# Autodesk Inventor assembly: 6_right_arm_no error
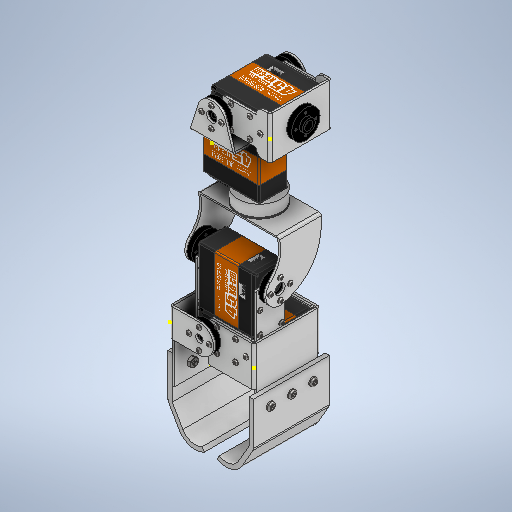
[picture p0: Inventor's stored thumbnail of the model, 512x512]
Saved by Autodesk Inventor 2026.1 (Build 301233000, 233)
## iProperties
Created: 2025-07-28
Part Number: 6_right_arm_no error
Document SubType Name: Assembly
Designer: LG
Author: LG
## Documents named in this file (20)
- C:\Users\LG\Desktop\RHp_Humanoid_ver1\Assembly\6_right_Arm.iam
- C:\Users\LG\Desktop\RHp_Humanoid_ver1\Part\HTD-45H, Horn\HTD-45H\HTD-45H.iam
- C:\Users\LG\Desktop\RHp_Humanoid_ver1\Part\HTD-45H, Horn\Horn\Top Horn.ipt
- C:\Users\LG\Desktop\RHp_Humanoid_ver1\Part\Frame\Arm\axis_18_top_frame.ipt
- C:\Users\LG\Desktop\RHp_Humanoid_ver1\Part\HTD-45H, Horn\Horn\Bottom Horn.ipt
- C:\Users\LG\Desktop\RHp_Humanoid_ver1\Part\Frame\Arm\axis_19_bottom_frame.ipt
- C:\Users\LG\Desktop\RHp_Humanoid_ver1\Part\Frame\Arm\axis_20_top_frame.ipt
- C:\Users\LG\Desktop\RHp_Humanoid_ver1\Part\Bolt, Bearing, Nut, Washer\2030 Teflon Sheet.ipt
- C:\Users\LG\Desktop\RHp_Humanoid_ver1\Part\Frame\Arm\axis_20_bottom_frame.ipt
- C:\Users\LG\Desktop\RHp_Humanoid_ver1\Part\Frame\Arm\axis_21_top_frame.ipt
- C:\Users\LG\Desktop\RHp_Humanoid_ver1\Part\Frame\Arm\axis_21_bottom_frame.ipt
- C:\Users\LG\Desktop\RHp_Humanoid_ver1\Part\Frame\Arm\axis_22_bottom_frame.ipt
- C:\Users\LG\Desktop\RHp_Humanoid_ver1\Part\Frame\Arm\axis_22_top_frame.ipt
- C:\Users\LG\Desktop\RHp_Humanoid_ver1\Part\Frame\Arm\HTD-45H_no bottom horn.ipt
- C:\Users\LG\Desktop\RHp_Humanoid_ver1\Part\Frame\Arm\gripper_frame.ipt
- C:\Users\LG\Desktop\RHp_Humanoid_ver1\Part\Bolt, Bearing, Nut, Washer\볼트, 너트\M2x4 Bolt.ipt
- C:\Users\LG\Desktop\RHp_Humanoid_ver1\Part\Bolt, Bearing, Nut, Washer\볼트, 너트\M3x6 Bolt.ipt
- C:\Users\LG\Desktop\RHp_Humanoid_ver1\Part\Bolt, Bearing, Nut, Washer\볼트, 너트\M3 Nut.ipt
- C:\Users\LG\Desktop\RHp_Humanoid_ver1\Part\Bolt, Bearing, Nut, Washer\볼트, 너트\M2x6 Bolt.ipt
- C:\Users\LG\Desktop\RHp_Humanoid_ver1\Part\Bolt, Bearing, Nut, Washer\볼트, 너트\M3x8 Bolt.ipt
## Components (107 placed, 18 different names)
1. M2x4 Bolt:21 — Rigid:22
2. M2x4 Bolt:20 — Rigid:21
3. M2x4 Bolt:19 — Rigid:20
4. M2x4 Bolt:18 — Rigid:19
5. M2x4 Bolt:6 — Rigid:6
6. M2x4 Bolt:8 — Rigid:2
7. M2x4 Bolt:7 — Rigid:3
8. M2x4 Bolt:9 — Rigid:4
9. M2x4 Bolt:1 — Rigid:5
10. M2x4 Bolt:10 — Rigid:12
11. M2x4 Bolt:11 — Rigid:13
12. M2x4 Bolt:17 — Rigid:11
13. M2x4 Bolt:16 — Rigid:14
14. axis_18_top_frame:1 — Mate:6, Mate:7, Mate:8, Mate:9, Mate:14, Mate:15, Rigid:2, Rigid:3, Rigid:4, Rigid:5, Rigid:6, Rigid:11, Rigid:12, Rigid:13, Rigid:14, Rigid:19, Rigid:20, Rigid:21, Rigid:22
15. Top Horn:1 — Mate:6, Mate:14, Mate:15
16. M2x4 Bolt:2 — Rigid:7
17. M2x4 Bolt:4 — Rigid:9
18. M2x4 Bolt:5 — Rigid:8
19. M2x4 Bolt:3 — Rigid:10
20. M2x4 Bolt:13 — Rigid:15
21. M2x4 Bolt:12 — Rigid:17
22. M2x4 Bolt:15 — Rigid:18
23. M2x4 Bolt:14 — Rigid:16
24. M2x4 Bolt:55 — Rigid:96
25. M2x4 Bolt:56 — Rigid:98
26. M2x4 Bolt:57 — Rigid:95
27. M2x4 Bolt:58 — Rigid:97
28. axis_19_bottom_frame:1 — Flush:2, Mate:12, Mate:13, Rigid:7, Rigid:8, Rigid:9, Rigid:10, Rigid:15, Rigid:16, Rigid:17, Rigid:18, Mate:49, Mate:50, Flush:15, Rigid:95, Rigid:96, Rigid:97, Rigid:98
29. Bottom Horn:1 — Mate:10, Mate:11, Flush:1
30. Top Horn:2 — Rotational:2, Flush:2, Mate:12, Mate:13
31. HTD-45H:2 [sub-assembly] — Mate:7, Mate:8, Mate:9, Rotational:2, Mate:10, Mate:11, Flush:1
32. 2030 Teflon Sheet:1 — Mate:19, Mate:20, Mate:21, Mate:24, Mate:25
33. 2030 Teflon Sheet:2 — Mate:24, Mate:25, Mate:26
34. M2x4 Bolt:27 — Rigid:27
35. M2x4 Bolt:28 — Rigid:29
36. M2x4 Bolt:29 — Rigid:30
37. M2x4 Bolt:26 — Rigid:28
38. axis_20_top_frame:1 — Mate:19, Mate:20, Mate:21, Mate:47, Flush:14, Mate:48
39. axis_20_bottom_frame:1 — Mate:22, Flush:6, Mate:23, Mate:26, Mate:29, Mate:30, Mate:31, Rigid:27, Rigid:28, Rigid:29, Rigid:30, Rigid:31, Rigid:32, Rigid:33, Rigid:34, Rigid:35, Rigid:36, Rigid:37, Rigid:38
40. Top Horn:3 — Mate:22, Flush:6, Mate:23, Rotational:6
41. HTD-45H:6 — Rotational:6, Mate:47, Flush:14, Mate:48, Mate:49, Mate:50, Flush:15
42. M2x4 Bolt:30 — Rigid:31
43. M2x4 Bolt:31 — Rigid:32
44. M2x4 Bolt:33 — Rigid:33
45. M2x4 Bolt:32 — Rigid:34
46. M2x4 Bolt:34 — Rigid:35
47. M2x4 Bolt:35 — Rigid:37
48. M2x4 Bolt:36 — Rigid:36
49. M2x4 Bolt:37 — Rigid:38
50. M2x4 Bolt:43 — Rigid:44
51. M2x4 Bolt:44 — Rigid:45
52. M2x4 Bolt:45 — Rigid:46
53. M2x4 Bolt:46 — Rigid:47
54. M2x4 Bolt:39 — Rigid:40
55. M2x4 Bolt:38 — Rigid:39
56. M2x4 Bolt:41 — Rigid:42
57. M2x4 Bolt:40 — Rigid:41
58. M2x4 Bolt:42 — Rigid:43
59. M3 Nut:3 — Rigid:64
60. M3 Nut:4 — Rigid:62
61. M3 Nut:2 — Rigid:63
62. M3 Nut:1 — Rigid:61
63. M3x6 Bolt:1 — Rigid:58
64. M3x6 Bolt:2 — Rigid:59
65. M3x6 Bolt:3 — Rigid:60
66. M3x6 Bolt:4 — Rigid:57
67. axis_21_top_frame:1 — Mate:36, Mate:37, Mate:38, Mate:39, Mate:45, Rigid:39, Rigid:40, Rigid:41, Rigid:42, Rigid:43, Rigid:44, Rigid:45, Rigid:46, Rigid:47, Rigid:57, Rigid:58, Rigid:59, Rigid:60
68. axis_21_bottom_frame:1 — Mate:39, Mate:40, Flush:10, Mate:44, Flush:11, Rigid:61, Rigid:62, Rigid:63, Rigid:64
69. Bottom Horn:2 — Mate:27, Flush:7, Mate:28
70. Top Horn:4 — Rotational:4, Mate:29, Mate:30, Mate:31
71. HTD-45H:4 [sub-assembly] — Mate:27, Flush:7, Mate:28, Rotational:4, Mate:35, Flush:8, Flush:9, Mate:37, Mate:38
72. M2x4 Bolt:47 — Rigid:65
73. M2x4 Bolt:49 — Rigid:66
74. M2x4 Bolt:50 — Rigid:68
75. M2x4 Bolt:48 — Rigid:67
76. M2x4 Bolt:54 — Rigid:69
77. M2x4 Bolt:51 — Rigid:70
78. M2x4 Bolt:53 — Rigid:72
79. M2x4 Bolt:52 — Rigid:71
80. M2x6 Bolt:5 — Rigid:77
81. M2x6 Bolt:7 — Rigid:78
82. M2x6 Bolt:6 — Rigid:79
83. M2x6 Bolt:8 — Rigid:80
84. M2x6 Bolt:9 — Rigid:81
85. M2x6 Bolt:2 — Rigid:74
86. M2x6 Bolt:1 — Rigid:73
87. M2x6 Bolt:3 — Rigid:76
88. M2x6 Bolt:4 — Rigid:75
89. M3x8 Bolt:4 — Rigid:88
90. M3x8 Bolt:5 — Rigid:89
91. M3x8 Bolt:6 — Rigid:90
92. M3 Nut:10 — Rigid:93
93. M3 Nut:9 — Rigid:92
94. M3 Nut:8 — Rigid:91
95. M3x8 Bolt:3 — Rigid:84
96. M3x8 Bolt:2 — Rigid:83
97. M3x8 Bolt:1 — Rigid:82
98. M3 Nut:6 — Rigid:87
99. M3 Nut:7 — Rigid:86
100. M3 Nut:5 — Rigid:85
101. axis_22_bottom_frame:1 — Mate:41, Mate:42, Mate:43, Rigid:1, Rigid:65, Rigid:66, Rigid:67, Rigid:68, Rigid:69, Rigid:70, Rigid:71, Rigid:72, Rigid:85, Rigid:86, Rigid:87
102. axis_22_top_frame:1 — Mate:44, Flush:11, Mate:45, Rigid:73, Rigid:74, Rigid:75, Rigid:76, Rigid:77, Rigid:78, Rigid:79, Rigid:80, Rigid:81, Rigid:91, Rigid:92, Rigid:93, Rigid:94
103. gripper_frame:1 — Rigid:1, Rigid:82, Rigid:83, Rigid:84
104. gripper_frame:2 — Rigid:88, Rigid:89, Rigid:90, Rigid:94
105. Top Horn:5 — Rotational:5, Mate:41, Mate:42, Mate:43
106. Bottom Horn:3 — Mate:32, Mate:33, Mate:34
107. HTD-45H:5 [sub-assembly] — Rotational:5, Mate:32, Mate:33, Mate:34, Mate:35, Flush:8, Flush:9, Mate:36, Mate:40, Flush:10
## Relationships (140: WeldJoint 85, Mate 41, Flush 10, RevoluteJoint 4)
- Rotational:2 [RevoluteJoint]: Top Horn:2 ↔ HTD-45H:2
- Rotational:4 [RevoluteJoint]: Top Horn:4 ↔ HTD-45H:4
- Rotational:5 [RevoluteJoint]: Top Horn:5 ↔ HTD-45H:5
- Rotational:6 [RevoluteJoint]: Top Horn:3 ↔ HTD-45H:6
- Mate:6: axis_18_top_frame:1 ↔ Top Horn:1
- Mate:7: axis_18_top_frame:1 ↔ HTD-45H:2
- Mate:8 (2.5 mm): axis_18_top_frame:1 ↔ HTD-45H:2
- Mate:9: axis_18_top_frame:1 ↔ HTD-45H:2
- Mate:10: Bottom Horn:1 ↔ HTD-45H:2
- Mate:11: Bottom Horn:1 ↔ HTD-45H:2
- Flush:1: Bottom Horn:1 ↔ HTD-45H:2
- Flush:2 (14.5 mm): axis_19_bottom_frame:1 ↔ Top Horn:2
- Mate:12: axis_19_bottom_frame:1 ↔ Top Horn:2
- Mate:13: axis_19_bottom_frame:1 ↔ Top Horn:2
- Mate:14: axis_18_top_frame:1 ↔ Top Horn:1
- Mate:15: axis_18_top_frame:1 ↔ Top Horn:1
- Mate:19: 2030 Teflon Sheet:1 ↔ axis_20_top_frame:1
- Mate:20: 2030 Teflon Sheet:1 ↔ axis_20_top_frame:1
- Mate:21: 2030 Teflon Sheet:1 ↔ axis_20_top_frame:1
- Mate:22: axis_20_bottom_frame:1 ↔ Top Horn:3
- Flush:6: axis_20_bottom_frame:1 ↔ Top Horn:3
- Mate:23: axis_20_bottom_frame:1 ↔ Top Horn:3
- Mate:24: 2030 Teflon Sheet:1 ↔ 2030 Teflon Sheet:2
- Mate:25: 2030 Teflon Sheet:1 ↔ 2030 Teflon Sheet:2
- Mate:26: 2030 Teflon Sheet:2 ↔ axis_20_bottom_frame:1
- Mate:27: Bottom Horn:2 ↔ HTD-45H:4
- Flush:7: Bottom Horn:2 ↔ HTD-45H:4
- Mate:28: Bottom Horn:2 ↔ HTD-45H:4
- Mate:29 (30.43 mm): axis_20_bottom_frame:1 ↔ Top Horn:4
- Mate:30 (-14 mm): axis_20_bottom_frame:1 ↔ Top Horn:4
- Mate:31: axis_20_bottom_frame:1 ↔ Top Horn:4
- Mate:32: Bottom Horn:3 ↔ HTD-45H:5
- Mate:33: Bottom Horn:3 ↔ HTD-45H:5
- Mate:34: Bottom Horn:3 ↔ HTD-45H:5
- Mate:35: HTD-45H:4 ↔ HTD-45H:5
- Flush:8: HTD-45H:4 ↔ HTD-45H:5
- Flush:9: HTD-45H:4 ↔ HTD-45H:5
- Mate:36 (5 mm): axis_21_top_frame:1 ↔ HTD-45H:5
- Mate:37: axis_21_top_frame:1 ↔ HTD-45H:4
- Mate:38: axis_21_top_frame:1 ↔ HTD-45H:4
- Mate:39: axis_21_top_frame:1 ↔ axis_21_bottom_frame:1
- Mate:40: axis_21_bottom_frame:1 ↔ HTD-45H:5
- Flush:10: axis_21_bottom_frame:1 ↔ HTD-45H:5
- Mate:41: axis_22_bottom_frame:1 ↔ Top Horn:5
- Mate:42: axis_22_bottom_frame:1 ↔ Top Horn:5
- Mate:43 (19.43 mm): axis_22_bottom_frame:1 ↔ Top Horn:5
- Mate:44: axis_21_bottom_frame:1 ↔ axis_22_top_frame:1
- Flush:11: axis_21_bottom_frame:1 ↔ axis_22_top_frame:1
- Mate:45: axis_21_top_frame:1 ↔ axis_22_top_frame:1
- Mate:47: axis_20_top_frame:1 ↔ HTD-45H:6
- Flush:14: axis_20_top_frame:1 ↔ HTD-45H:6
- Mate:48: axis_20_top_frame:1 ↔ HTD-45H:6
- Rigid:1 [WeldJoint]: axis_22_bottom_frame:1 ↔ gripper_frame:1
- Rigid:2 [WeldJoint]: M2x4 Bolt:8 ↔ axis_18_top_frame:1
- Rigid:3 [WeldJoint]: M2x4 Bolt:7 ↔ axis_18_top_frame:1
- Rigid:4 [WeldJoint]: M2x4 Bolt:9 ↔ axis_18_top_frame:1
- Rigid:5 [WeldJoint]: M2x4 Bolt:1 ↔ axis_18_top_frame:1
- Rigid:6 [WeldJoint]: M2x4 Bolt:6 ↔ axis_18_top_frame:1
- Rigid:7 [WeldJoint]: M2x4 Bolt:2 ↔ axis_19_bottom_frame:1
- Rigid:8 [WeldJoint]: M2x4 Bolt:5 ↔ axis_19_bottom_frame:1
- Rigid:9 [WeldJoint]: M2x4 Bolt:4 ↔ axis_19_bottom_frame:1
- Rigid:10 [WeldJoint]: M2x4 Bolt:3 ↔ axis_19_bottom_frame:1
- Rigid:11 [WeldJoint]: M2x4 Bolt:17 ↔ axis_18_top_frame:1
- Rigid:12 [WeldJoint]: M2x4 Bolt:10 ↔ axis_18_top_frame:1
- Rigid:13 [WeldJoint]: M2x4 Bolt:11 ↔ axis_18_top_frame:1
- Rigid:14 [WeldJoint]: M2x4 Bolt:16 ↔ axis_18_top_frame:1
- Rigid:15 [WeldJoint]: M2x4 Bolt:13 ↔ axis_19_bottom_frame:1
- Rigid:16 [WeldJoint]: M2x4 Bolt:14 ↔ axis_19_bottom_frame:1
- Rigid:17 [WeldJoint]: M2x4 Bolt:12 ↔ axis_19_bottom_frame:1
- Rigid:18 [WeldJoint]: M2x4 Bolt:15 ↔ axis_19_bottom_frame:1
- Rigid:19 [WeldJoint]: M2x4 Bolt:18 ↔ axis_18_top_frame:1
- Rigid:20 [WeldJoint]: M2x4 Bolt:19 ↔ axis_18_top_frame:1
- Rigid:21 [WeldJoint]: M2x4 Bolt:20 ↔ axis_18_top_frame:1
- Rigid:22 [WeldJoint]: M2x4 Bolt:21 ↔ axis_18_top_frame:1
- Rigid:27 [WeldJoint]: M2x4 Bolt:27 ↔ axis_20_bottom_frame:1
- Rigid:28 [WeldJoint]: M2x4 Bolt:26 ↔ axis_20_bottom_frame:1
- Rigid:29 [WeldJoint]: M2x4 Bolt:28 ↔ axis_20_bottom_frame:1
- Rigid:30 [WeldJoint]: M2x4 Bolt:29 ↔ axis_20_bottom_frame:1
- Rigid:31 [WeldJoint]: axis_20_bottom_frame:1 ↔ M2x4 Bolt:30
- Rigid:32 [WeldJoint]: axis_20_bottom_frame:1 ↔ M2x4 Bolt:31
- Rigid:33 [WeldJoint]: axis_20_bottom_frame:1 ↔ M2x4 Bolt:33
- Rigid:34 [WeldJoint]: axis_20_bottom_frame:1 ↔ M2x4 Bolt:32
- Rigid:35 [WeldJoint]: axis_20_bottom_frame:1 ↔ M2x4 Bolt:34
- Rigid:36 [WeldJoint]: axis_20_bottom_frame:1 ↔ M2x4 Bolt:36
- Rigid:37 [WeldJoint]: axis_20_bottom_frame:1 ↔ M2x4 Bolt:35
- Rigid:38 [WeldJoint]: axis_20_bottom_frame:1 ↔ M2x4 Bolt:37
- Rigid:39 [WeldJoint]: M2x4 Bolt:38 ↔ axis_21_top_frame:1
- Rigid:40 [WeldJoint]: M2x4 Bolt:39 ↔ axis_21_top_frame:1
- Rigid:41 [WeldJoint]: M2x4 Bolt:40 ↔ axis_21_top_frame:1
- Rigid:42 [WeldJoint]: M2x4 Bolt:41 ↔ axis_21_top_frame:1
- Rigid:43 [WeldJoint]: M2x4 Bolt:42 ↔ axis_21_top_frame:1
- Rigid:44 [WeldJoint]: M2x4 Bolt:43 ↔ axis_21_top_frame:1
- Rigid:45 [WeldJoint]: M2x4 Bolt:44 ↔ axis_21_top_frame:1
- Rigid:46 [WeldJoint]: M2x4 Bolt:45 ↔ axis_21_top_frame:1
- Rigid:47 [WeldJoint]: M2x4 Bolt:46 ↔ axis_21_top_frame:1
- Rigid:57 [WeldJoint]: M3x6 Bolt:4 ↔ axis_21_top_frame:1
- Rigid:58 [WeldJoint]: M3x6 Bolt:1 ↔ axis_21_top_frame:1
- Rigid:59 [WeldJoint]: M3x6 Bolt:2 ↔ axis_21_top_frame:1
- Rigid:60 [WeldJoint]: M3x6 Bolt:3 ↔ axis_21_top_frame:1
- Rigid:61 [WeldJoint]: M3 Nut:1 ↔ axis_21_bottom_frame:1
- Rigid:62 [WeldJoint]: M3 Nut:4 ↔ axis_21_bottom_frame:1
- Rigid:63 [WeldJoint]: M3 Nut:2 ↔ axis_21_bottom_frame:1
- Rigid:64 [WeldJoint]: M3 Nut:3 ↔ axis_21_bottom_frame:1
- Rigid:65 [WeldJoint]: M2x4 Bolt:47 ↔ axis_22_bottom_frame:1
- Rigid:66 [WeldJoint]: M2x4 Bolt:49 ↔ axis_22_bottom_frame:1
- Rigid:67 [WeldJoint]: M2x4 Bolt:48 ↔ axis_22_bottom_frame:1
- Rigid:68 [WeldJoint]: M2x4 Bolt:50 ↔ axis_22_bottom_frame:1
- Rigid:69 [WeldJoint]: M2x4 Bolt:54 ↔ axis_22_bottom_frame:1
- Rigid:70 [WeldJoint]: M2x4 Bolt:51 ↔ axis_22_bottom_frame:1
- Rigid:71 [WeldJoint]: M2x4 Bolt:52 ↔ axis_22_bottom_frame:1
- Rigid:72 [WeldJoint]: M2x4 Bolt:53 ↔ axis_22_bottom_frame:1
- Rigid:73 [WeldJoint]: M2x6 Bolt:1 ↔ axis_22_top_frame:1
- Rigid:74 [WeldJoint]: M2x6 Bolt:2 ↔ axis_22_top_frame:1
- Rigid:75 [WeldJoint]: M2x6 Bolt:4 ↔ axis_22_top_frame:1
- Rigid:76 [WeldJoint]: M2x6 Bolt:3 ↔ axis_22_top_frame:1
- Rigid:77 [WeldJoint]: M2x6 Bolt:5 ↔ axis_22_top_frame:1
- Rigid:78 [WeldJoint]: M2x6 Bolt:7 ↔ axis_22_top_frame:1
- Rigid:79 [WeldJoint]: M2x6 Bolt:6 ↔ axis_22_top_frame:1
- Rigid:80 [WeldJoint]: M2x6 Bolt:8 ↔ axis_22_top_frame:1
- Rigid:81 [WeldJoint]: M2x6 Bolt:9 ↔ axis_22_top_frame:1
- Rigid:82 [WeldJoint]: M3x8 Bolt:1 ↔ gripper_frame:1
- Rigid:83 [WeldJoint]: M3x8 Bolt:2 ↔ gripper_frame:1
- Rigid:84 [WeldJoint]: M3x8 Bolt:3 ↔ gripper_frame:1
- Rigid:85 [WeldJoint]: M3 Nut:5 ↔ axis_22_bottom_frame:1
- Rigid:86 [WeldJoint]: M3 Nut:7 ↔ axis_22_bottom_frame:1
- Rigid:87 [WeldJoint]: M3 Nut:6 ↔ axis_22_bottom_frame:1
- Rigid:88 [WeldJoint]: M3x8 Bolt:4 ↔ gripper_frame:2
- Rigid:89 [WeldJoint]: M3x8 Bolt:5 ↔ gripper_frame:2
- Rigid:90 [WeldJoint]: M3x8 Bolt:6 ↔ gripper_frame:2
- Rigid:91 [WeldJoint]: M3 Nut:8 ↔ axis_22_top_frame:1
- Rigid:92 [WeldJoint]: M3 Nut:9 ↔ axis_22_top_frame:1
- Rigid:93 [WeldJoint]: M3 Nut:10 ↔ axis_22_top_frame:1
- Rigid:94 [WeldJoint]: axis_22_top_frame:1 ↔ gripper_frame:2
- Mate:49: axis_19_bottom_frame:1 ↔ HTD-45H:6
- Mate:50: axis_19_bottom_frame:1 ↔ HTD-45H:6
- Flush:15: axis_19_bottom_frame:1 ↔ HTD-45H:6
- Rigid:95 [WeldJoint]: M2x4 Bolt:57 ↔ axis_19_bottom_frame:1
- Rigid:96 [WeldJoint]: M2x4 Bolt:55 ↔ axis_19_bottom_frame:1
- Rigid:97 [WeldJoint]: M2x4 Bolt:58 ↔ axis_19_bottom_frame:1
- Rigid:98 [WeldJoint]: M2x4 Bolt:56 ↔ axis_19_bottom_frame:1
